# Autodesk Inventor assembly: Assembly9 (Crank Case Sub Assembly)
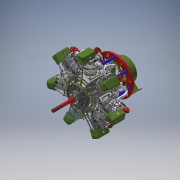
[picture p0: Inventor's stored thumbnail of the model, 180x180]
Saved by Autodesk Inventor 2018 (Build 220112000, 112)
## iProperties
Created: 2023-05-02
Part Number: Assembly9 (Crank Case Sub Assembly)
Document SubType Name: Assembly
Designer: Habib Mohamed
Author: Habib Mohamed
## Documents named in this file (19)
- D:\Inventor\My projects\Rotary Engine\Assembly\Assembly9 (Crank Case Sub Assembly).iam
- D:\Inventor\My projects\Rotary Engine\Main Block (Crank Case).ipt
- D:\Inventor\My projects\Rotary Engine\Assembly\Assembly8 (Cylinder Complete Sub Assembly).iam
- D:\Inventor\My projects\Rotary Engine\Assembly\Assembly6(Piston Sub Assembly Major).iam
- C:\Users\Habib Mohamed\Documents\Inventor\Content Center Files\R2018\en-US\ISO 4762(1)\DIN EN ISO 4762 - M4 x 12.ipt
- D:\Inventor\My projects\Rotary Engine\Assembly\Assembly10(Suction houe sub assembly).iam
- D:\Inventor\My projects\Rotary Engine\Component 9 (Suspension Spacer).ipt
- D:\Inventor\My projects\Rotary Engine\Component 10(Assembly Ring).ipt
- D:\Inventor\My projects\Rotary Engine\Assembly\Exhaust Pipe Sub-Assembly.iam
- D:\Inventor\My projects\Rotary Engine\Assembly\Assembly2 (Intake Pipe Sub Assembly).iam
- D:\Inventor\My projects\Rotary Engine\Component 46(Engine Gas Collector).ipt
- C:\Users\Habib Mohamed\Documents\Inventor\Content Center Files\R2018\en-US\ISO 4762(1)\DIN EN ISO 4762 - M3 x 5.ipt
- C:\Users\Habib Mohamed\Documents\Inventor\Content Center Files\R2018\en-US\ISO 4762(1)\DIN EN ISO 4762 - M4 x 8.ipt
- C:\Users\Habib Mohamed\Documents\Inventor\Content Center Files\R2018\en-US\ISO 10511\ISO 10511 - M5.ipt
- D:\Inventor\My projects\Rotary Engine\Assembly\Assembly11 (Cam Sub Assembly).iam
- D:\Inventor\My projects\Rotary Engine\Component 20 (Planet Wheel).ipt
- D:\Inventor\My projects\Rotary Engine\Component 3 (Planet Gear Axis).ipt
- C:\Users\Habib Mohamed\Documents\Inventor\Content Center Files\R2018\en-US\DIN 618 - T1  HK\DIN 618 - HK0609 - 6 x 10 x 9.ipt
- C:\Users\Habib Mohamed\Documents\Inventor\Content Center Files\R2018\en-US\DIN 6799\DIN 6799 - 6 7.ipt
## Components (116 placed, 18 different names)
1. Main Block (Crank Case):1 — Mate:1, Mate:2, Mate:3, Mate:4, Mate:6, Mate:7, Mate:8, Mate:9, Mate:10, Mate:11, Mate:12, Mate:13, Mate:14, Mate:16, Mate:18, Mate:20, Mate:22, Mate:23, Mate:24, Mate:25, Mate:26, Mate:27, Mate:28, Mate:37, Mate:48, Mate:50, Mate:52, Mate:54, Mate:56, Mate:58, Mate:60, Mate:65, Mate:66, Mate:67, Mate:68, Mate:69, Mate:70, Mate:74, Mate:75, Mate:76, Mate:90
2. Assembly6(Piston Sub Assembly Major):1 [sub-assembly] — Mate:1, Mate:5, Mate:6, Mate:7, Mate:8, Mate:9, Mate:10, Mate:11, Mate:12, Mate:89
3. Assembly10(Suction houe sub assembly):1 [sub-assembly] — Mate:23, Mate:24, Mate:25, Mate:49, Mate:51, Mate:53, Mate:55, Mate:57, Mate:59, Mate:61
4. Component 10(Assembly Ring):1 — Mate:28, Mate:29, Mate:30, Mate:63
5. Component 46(Engine Gas Collector):1 — Mate:37, Mate:38, Mate:39, Mate:64
6. DIN EN ISO 4762 M4 x 8:1 — Mate:48, Mate:49
7. DIN EN ISO 4762 M4 x 8:2 — Mate:50, Mate:51
8. DIN EN ISO 4762 M4 x 8:3 — Mate:52, Mate:53
9. DIN EN ISO 4762 M4 x 8:4 — Mate:54, Mate:55
10. DIN EN ISO 4762 M4 x 8:5 — Mate:56, Mate:57
11. DIN EN ISO 4762 M4 x 8:6 — Mate:58, Mate:59
12. DIN EN ISO 4762 M4 x 8:7 — Mate:60, Mate:61
13. Assembly11 (Cam Sub Assembly):1 [sub-assembly] — Mate:89, Mate:90, Tangent:1, Tangent:2
14. Component 20 (Planet Wheel):1 — Mate:72, Mate:76
15. Component 20 (Planet Wheel):2 — Mate:73, Mate:74
16. Component 20 (Planet Wheel):3 — Mate:71, Mate:75
17. Component 3 (Planet Gear Axis):1 — Mate:65, Mate:68, Mate:71, Mate:79, Mate:80, Mate:85
18. Component 3 (Planet Gear Axis):2 — Mate:67, Mate:70, Mate:72, Mate:77, Mate:78, Mate:87
19. Component 3 (Planet Gear Axis):3 — Mate:66, Mate:69, Mate:73, Mate:81, Mate:82, Mate:83
20. DIN 618 - T1 HK HK0609 - 6 x 10 x 9:1 — Mate:77, Mate:78, Mate:88
21. DIN 618 - T1 HK HK0609 - 6 x 10 x 9:2 — Mate:79, Mate:80, Mate:86
22. DIN 618 - T1 HK HK0609 - 6 x 10 x 9:3 — Mate:81, Mate:82, Mate:84
23. DIN 6799 6:1 — Mate:83, Mate:84
24. DIN 6799 6:2 — Mate:85, Mate:86
25. DIN 6799 6:3 — Mate:87, Mate:88
26. Assembly8 (Cylinder Complete Sub Assembly):1 [sub-assembly] — Mate:2, Mate:3, Mate:4, Mate:5, Mate:13, Mate:15, Mate:17, Mate:19, Mate:21
27. DIN EN ISO 4762 M4 x 12:1 — Mate:14, Mate:15
28. DIN EN ISO 4762 M4 x 12:2 — Mate:16, Mate:17
29. DIN EN ISO 4762 M4 x 12:3 — Mate:18, Mate:19
30. DIN EN ISO 4762 M4 x 12:4 — Mate:20, Mate:21
31. Assembly8 (Cylinder Complete Sub Assembly):2 [sub-assembly]
32. DIN EN ISO 4762 M4 x 12:5
33. DIN EN ISO 4762 M4 x 12:6
34. DIN EN ISO 4762 M4 x 12:7
35. DIN EN ISO 4762 M4 x 12:8
36. Assembly8 (Cylinder Complete Sub Assembly):3 [sub-assembly]
37. DIN EN ISO 4762 M4 x 12:9
38. DIN EN ISO 4762 M4 x 12:10
39. DIN EN ISO 4762 M4 x 12:11
40. DIN EN ISO 4762 M4 x 12:12
41. Assembly8 (Cylinder Complete Sub Assembly):4 [sub-assembly]
42. DIN EN ISO 4762 M4 x 12:13
43. DIN EN ISO 4762 M4 x 12:14
44. DIN EN ISO 4762 M4 x 12:15
45. DIN EN ISO 4762 M4 x 12:16
46. Assembly8 (Cylinder Complete Sub Assembly):5 [sub-assembly] — Mate:31, Mate:32, Mate:33, Mate:34, Mate:35, Mate:36, Mate:40, Mate:42, Mate:44, Mate:46, Tangent:1, Tangent:2
47. DIN EN ISO 4762 M4 x 12:17
48. DIN EN ISO 4762 M4 x 12:18
49. DIN EN ISO 4762 M4 x 12:19
50. DIN EN ISO 4762 M4 x 12:20
51. Assembly8 (Cylinder Complete Sub Assembly):6 [sub-assembly]
52. DIN EN ISO 4762 M4 x 12:21
53. DIN EN ISO 4762 M4 x 12:22
54. DIN EN ISO 4762 M4 x 12:23
55. DIN EN ISO 4762 M4 x 12:24
56. Assembly8 (Cylinder Complete Sub Assembly):7 [sub-assembly]
57. DIN EN ISO 4762 M4 x 12:25
58. DIN EN ISO 4762 M4 x 12:26
59. DIN EN ISO 4762 M4 x 12:27
60. DIN EN ISO 4762 M4 x 12:28
61. DIN EN ISO 4762 M3 x 5:2 — Mate:42, Mate:43
62. DIN EN ISO 4762 M3 x 5:1 — Mate:40, Mate:41
63. Assembly2 (Intake Pipe Sub Assembly):1 [sub-assembly] — Mate:31, Mate:32, Mate:33, Mate:41, Mate:43
64. Exhaust Pipe Sub-Assembly:1 [sub-assembly] — Mate:34, Mate:35, Mate:36, Mate:38, Mate:39, Mate:45, Mate:47
65. DIN EN ISO 4762 M3 x 5:3 — Mate:44, Mate:45
66. DIN EN ISO 4762 M3 x 5:4 — Mate:46, Mate:47
67. Component 9 (Suspension Spacer):1 — Mate:26, Mate:27, Mate:29, Mate:30, Mate:62
68. DIN EN ISO 10511 M5:1 — Mate:62, Mate:63
69. DIN EN ISO 4762 M3 x 5:5
70. DIN EN ISO 4762 M3 x 5:6
71. Assembly2 (Intake Pipe Sub Assembly):2 [sub-assembly]
72. Exhaust Pipe Sub-Assembly:2 [sub-assembly]
73. DIN EN ISO 4762 M3 x 5:7
74. DIN EN ISO 4762 M3 x 5:8
75. Component 9 (Suspension Spacer):2
76. DIN EN ISO 10511 M5:2
77. DIN EN ISO 4762 M3 x 5:9
78. DIN EN ISO 4762 M3 x 5:10
79. Assembly2 (Intake Pipe Sub Assembly):3 [sub-assembly]
80. Exhaust Pipe Sub-Assembly:3 [sub-assembly]
81. DIN EN ISO 4762 M3 x 5:11
82. DIN EN ISO 4762 M3 x 5:12
83. Component 9 (Suspension Spacer):3
84. DIN EN ISO 10511 M5:3
85. DIN EN ISO 4762 M3 x 5:13
86. DIN EN ISO 4762 M3 x 5:14
87. Assembly2 (Intake Pipe Sub Assembly):4 [sub-assembly]
88. Exhaust Pipe Sub-Assembly:4 [sub-assembly]
89. DIN EN ISO 4762 M3 x 5:15
90. DIN EN ISO 4762 M3 x 5:16
91. Component 9 (Suspension Spacer):4
92. DIN EN ISO 10511 M5:4
93. DIN EN ISO 4762 M3 x 5:17
94. DIN EN ISO 4762 M3 x 5:18
95. Assembly2 (Intake Pipe Sub Assembly):5 [sub-assembly]
96. Exhaust Pipe Sub-Assembly:5 [sub-assembly]
97. DIN EN ISO 4762 M3 x 5:19
98. DIN EN ISO 4762 M3 x 5:20
99. Component 9 (Suspension Spacer):5
100. DIN EN ISO 10511 M5:5
101. DIN EN ISO 4762 M3 x 5:21
102. DIN EN ISO 4762 M3 x 5:22
103. Assembly2 (Intake Pipe Sub Assembly):6 [sub-assembly]
104. Exhaust Pipe Sub-Assembly:6 [sub-assembly]
105. DIN EN ISO 4762 M3 x 5:23
106. DIN EN ISO 4762 M3 x 5:24
107. Component 9 (Suspension Spacer):6
108. DIN EN ISO 10511 M5:6
109. DIN EN ISO 4762 M3 x 5:25
110. DIN EN ISO 4762 M3 x 5:26
111. Assembly2 (Intake Pipe Sub Assembly):7 [sub-assembly]
112. Exhaust Pipe Sub-Assembly:7 [sub-assembly]
113. DIN EN ISO 4762 M3 x 5:27
114. DIN EN ISO 4762 M3 x 5:28
115. Component 9 (Suspension Spacer):7
116. DIN EN ISO 10511 M5:7
## Component patterns: (7 elements, first: Assembly8 (Cylinder Complete Sub Assembly):1 + DIN EN ISO 4762 M4 x 12:1 + DIN EN ISO 4762 M4 x 12:2 + DIN EN ISO 4762 M4 x 12:3 + DIN EN ISO 4762 M4 x 12:4), (7 elements, first: DIN EN ISO 4762 M3 x 5:2 + DIN EN ISO 4762 M3 x 5:1 + Assembly2 (Intake Pipe Sub Assembly):1 + Exhaust Pipe Sub-Assembly:1 + DIN EN ISO 4762 M3 x 5:3 + DIN EN ISO 4762 M3 x 5:4 + Component 9 (Suspension Spacer):1 + DIN EN ISO 10511 M5:1)
## Relationships (92: Mate 90, Tangent 2)
- Mate:1: Main Block (Crank Case):1 ↔ Assembly6(Piston Sub Assembly Major):1
- Mate:2: Main Block (Crank Case):1 ↔ Assembly8 (Cylinder Complete Sub Assembly):1
- Mate:3: Main Block (Crank Case):1 ↔ Assembly8 (Cylinder Complete Sub Assembly):1
- Mate:4: Main Block (Crank Case):1 ↔ Assembly8 (Cylinder Complete Sub Assembly):1
- Mate:5: Assembly6(Piston Sub Assembly Major):1 ↔ Assembly8 (Cylinder Complete Sub Assembly):1
- Mate:6: Main Block (Crank Case):1 ↔ Assembly6(Piston Sub Assembly Major):1
- Mate:7: Main Block (Crank Case):1 ↔ Assembly6(Piston Sub Assembly Major):1
- Mate:8: Main Block (Crank Case):1 ↔ Assembly6(Piston Sub Assembly Major):1
- Mate:9: Main Block (Crank Case):1 ↔ Assembly6(Piston Sub Assembly Major):1
- Mate:10: Main Block (Crank Case):1 ↔ Assembly6(Piston Sub Assembly Major):1
- Mate:11: Main Block (Crank Case):1 ↔ Assembly6(Piston Sub Assembly Major):1
- Mate:12: Main Block (Crank Case):1 ↔ Assembly6(Piston Sub Assembly Major):1
- Mate:13: Main Block (Crank Case):1 ↔ Assembly8 (Cylinder Complete Sub Assembly):1
- Mate:14: Main Block (Crank Case):1 ↔ DIN EN ISO 4762 M4 x 12:1
- Mate:15: Assembly8 (Cylinder Complete Sub Assembly):1 ↔ DIN EN ISO 4762 M4 x 12:1
- Mate:16: Main Block (Crank Case):1 ↔ DIN EN ISO 4762 M4 x 12:2
- Mate:17: Assembly8 (Cylinder Complete Sub Assembly):1 ↔ DIN EN ISO 4762 M4 x 12:2
- Mate:18: Main Block (Crank Case):1 ↔ DIN EN ISO 4762 M4 x 12:3
- Mate:19: Assembly8 (Cylinder Complete Sub Assembly):1 ↔ DIN EN ISO 4762 M4 x 12:3
- Mate:20: Main Block (Crank Case):1 ↔ DIN EN ISO 4762 M4 x 12:4
- Mate:21: Assembly8 (Cylinder Complete Sub Assembly):1 ↔ DIN EN ISO 4762 M4 x 12:4
- Mate:22: Main Block (Crank Case):1
- Mate:23: Main Block (Crank Case):1 ↔ Assembly10(Suction houe sub assembly):1
- Mate:24: Main Block (Crank Case):1 ↔ Assembly10(Suction houe sub assembly):1
- Mate:25: Main Block (Crank Case):1 ↔ Assembly10(Suction houe sub assembly):1
- Mate:26: Main Block (Crank Case):1 ↔ Component 9 (Suspension Spacer):1
- Mate:27: Main Block (Crank Case):1 ↔ Component 9 (Suspension Spacer):1
- Mate:28: Main Block (Crank Case):1 ↔ Component 10(Assembly Ring):1
- Mate:29: Component 10(Assembly Ring):1 ↔ Component 9 (Suspension Spacer):1
- Mate:30: Component 10(Assembly Ring):1 ↔ Component 9 (Suspension Spacer):1
- Mate:31: Assembly8 (Cylinder Complete Sub Assembly):5 ↔ Assembly2 (Intake Pipe Sub Assembly):1
- Mate:32: Assembly8 (Cylinder Complete Sub Assembly):5 ↔ Assembly2 (Intake Pipe Sub Assembly):1
- Mate:33: Assembly8 (Cylinder Complete Sub Assembly):5 ↔ Assembly2 (Intake Pipe Sub Assembly):1
- Mate:34: Assembly8 (Cylinder Complete Sub Assembly):5 ↔ Exhaust Pipe Sub-Assembly:1
- Mate:35: Assembly8 (Cylinder Complete Sub Assembly):5 ↔ Exhaust Pipe Sub-Assembly:1
- Mate:36: Assembly8 (Cylinder Complete Sub Assembly):5 ↔ Exhaust Pipe Sub-Assembly:1
- Mate:37: Main Block (Crank Case):1 ↔ Component 46(Engine Gas Collector):1
- Mate:38: Component 46(Engine Gas Collector):1 ↔ Exhaust Pipe Sub-Assembly:1
- Mate:39: Component 46(Engine Gas Collector):1 ↔ Exhaust Pipe Sub-Assembly:1
- Mate:40: Assembly8 (Cylinder Complete Sub Assembly):5 ↔ DIN EN ISO 4762 M3 x 5:1
- Mate:41: DIN EN ISO 4762 M3 x 5:1 ↔ Assembly2 (Intake Pipe Sub Assembly):1
- Mate:42: Assembly8 (Cylinder Complete Sub Assembly):5 ↔ DIN EN ISO 4762 M3 x 5:2
- Mate:43: DIN EN ISO 4762 M3 x 5:2 ↔ Assembly2 (Intake Pipe Sub Assembly):1
- Mate:44: Assembly8 (Cylinder Complete Sub Assembly):5 ↔ DIN EN ISO 4762 M3 x 5:3
- Mate:45: Exhaust Pipe Sub-Assembly:1 ↔ DIN EN ISO 4762 M3 x 5:3
- Mate:46: Assembly8 (Cylinder Complete Sub Assembly):5 ↔ DIN EN ISO 4762 M3 x 5:4
- Mate:47: Exhaust Pipe Sub-Assembly:1 ↔ DIN EN ISO 4762 M3 x 5:4
- Mate:48: Main Block (Crank Case):1 ↔ DIN EN ISO 4762 M4 x 8:1
- Mate:49: Assembly10(Suction houe sub assembly):1 ↔ DIN EN ISO 4762 M4 x 8:1
- Mate:50: Main Block (Crank Case):1 ↔ DIN EN ISO 4762 M4 x 8:2
- Mate:51: Assembly10(Suction houe sub assembly):1 ↔ DIN EN ISO 4762 M4 x 8:2
- Mate:52: Main Block (Crank Case):1 ↔ DIN EN ISO 4762 M4 x 8:3
- Mate:53: Assembly10(Suction houe sub assembly):1 ↔ DIN EN ISO 4762 M4 x 8:3
- Mate:54: Main Block (Crank Case):1 ↔ DIN EN ISO 4762 M4 x 8:4
- Mate:55: Assembly10(Suction houe sub assembly):1 ↔ DIN EN ISO 4762 M4 x 8:4
- Mate:56: Main Block (Crank Case):1 ↔ DIN EN ISO 4762 M4 x 8:5
- Mate:57: Assembly10(Suction houe sub assembly):1 ↔ DIN EN ISO 4762 M4 x 8:5
- Mate:58: Main Block (Crank Case):1 ↔ DIN EN ISO 4762 M4 x 8:6
- Mate:59: Assembly10(Suction houe sub assembly):1 ↔ DIN EN ISO 4762 M4 x 8:6
- Mate:60: Main Block (Crank Case):1 ↔ DIN EN ISO 4762 M4 x 8:7
- Mate:61: Assembly10(Suction houe sub assembly):1 ↔ DIN EN ISO 4762 M4 x 8:7
- Mate:62: Component 9 (Suspension Spacer):1 ↔ DIN EN ISO 10511 M5:1
- Mate:63: Component 10(Assembly Ring):1 ↔ DIN EN ISO 10511 M5:1
- Mate:64: Component 46(Engine Gas Collector):1
- Mate:65: Main Block (Crank Case):1 ↔ Component 3 (Planet Gear Axis):1
- Mate:66: Main Block (Crank Case):1 ↔ Component 3 (Planet Gear Axis):3
- Mate:67: Main Block (Crank Case):1 ↔ Component 3 (Planet Gear Axis):2
- Mate:68: Main Block (Crank Case):1 ↔ Component 3 (Planet Gear Axis):1
- Mate:69: Main Block (Crank Case):1 ↔ Component 3 (Planet Gear Axis):3
- Mate:70: Main Block (Crank Case):1 ↔ Component 3 (Planet Gear Axis):2
- Mate:71: Component 20 (Planet Wheel):3 ↔ Component 3 (Planet Gear Axis):1
- Mate:72: Component 20 (Planet Wheel):1 ↔ Component 3 (Planet Gear Axis):2
- Mate:73: Component 20 (Planet Wheel):2 ↔ Component 3 (Planet Gear Axis):3
- Mate:74: Main Block (Crank Case):1 ↔ Component 20 (Planet Wheel):2
- Mate:75: Main Block (Crank Case):1 ↔ Component 20 (Planet Wheel):3
- Mate:76: Main Block (Crank Case):1 ↔ Component 20 (Planet Wheel):1
- Mate:77: Component 3 (Planet Gear Axis):2 ↔ DIN 618 - T1 HK HK0609 - 6 x 10 x 9:1
- Mate:78: Component 3 (Planet Gear Axis):2 ↔ DIN 618 - T1 HK HK0609 - 6 x 10 x 9:1
- Mate:79: Component 3 (Planet Gear Axis):1 ↔ DIN 618 - T1 HK HK0609 - 6 x 10 x 9:2
- Mate:80: Component 3 (Planet Gear Axis):1 ↔ DIN 618 - T1 HK HK0609 - 6 x 10 x 9:2
- Mate:81: Component 3 (Planet Gear Axis):3 ↔ DIN 618 - T1 HK HK0609 - 6 x 10 x 9:3
- Mate:82: Component 3 (Planet Gear Axis):3 ↔ DIN 618 - T1 HK HK0609 - 6 x 10 x 9:3
- Mate:83: Component 3 (Planet Gear Axis):3 ↔ DIN 6799 6:1
- Mate:84: DIN 618 - T1 HK HK0609 - 6 x 10 x 9:3 ↔ DIN 6799 6:1
- Mate:85: Component 3 (Planet Gear Axis):1 ↔ DIN 6799 6:2
- Mate:86: DIN 618 - T1 HK HK0609 - 6 x 10 x 9:2 ↔ DIN 6799 6:2
- Mate:87: Component 3 (Planet Gear Axis):2 ↔ DIN 6799 6:3
- Mate:88: DIN 618 - T1 HK HK0609 - 6 x 10 x 9:1 ↔ DIN 6799 6:3
- Mate:89: Assembly6(Piston Sub Assembly Major):1 ↔ Assembly11 (Cam Sub Assembly):1
- Mate:90: Main Block (Crank Case):1 ↔ Assembly11 (Cam Sub Assembly):1
- Tangent:1: Assembly11 (Cam Sub Assembly):1 ↔ Assembly8 (Cylinder Complete Sub Assembly):5
- Tangent:2: Assembly11 (Cam Sub Assembly):1 ↔ Assembly8 (Cylinder Complete Sub Assembly):5
